# Autodesk Inventor assembly: Upper Stage
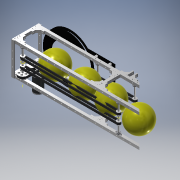
[picture p0: Inventor's stored thumbnail of the model, 180x180]
Saved by Autodesk Inventor 2019.4 (Build 234330000, 330)
## iProperties
Created: 2020-01-18
Part Number: Upper Stage
Document SubType Name: Assembly
Designer: Mark
Mass: 13649.7 g
Surface Area: 29206.4 cm^2
Volume: 17282.3 cm^3
Density: 0.789809 g/cm^3
Author: Mark
## Documents named in this file (21)
- C:\Users\admin\Desktop\FRC 2020 Engineering\GitHub\7738-2020\Upper Stage\Upper Stage.iam
- C:\Users\admin\Desktop\FRC 2020 Engineering\GitHub\7738-2020\Upper Stage\Main Extrusions.ipt
- C:\Users\admin\Desktop\FRC 2020 Engineering\GitHub\7738-2020\Upper Stage\Secondary Extrusions.ipt
- C:\Users\admin\Desktop\FRC 2020 Engineering\GitHub\7738-2020\Power Cell.ipt
- C:\Users\admin\Desktop\FRC 2020 Engineering\GitHub\7738-2020\Upper Stage\First stage shaft.ipt
- C:\Users\admin\Desktop\FRC 2020 Engineering\GitHub\7738-2020\Upper Stage\KFL08.ipt
- C:\Users\admin\Desktop\FRC 2020 Engineering\GitHub\7738-2020\Upper Stage\Turret Support.ipt
- C:\Users\admin\Desktop\FRC 2020 Engineering\GitHub\7738-2020\Upper Stage\HTD 5M 15 Teeth.ipt
- C:\Users\admin\Desktop\FRC 2020 Engineering\GitHub\7738-2020\Upper Stage\HTD 5M 775.ipt
- C:\Users\admin\Desktop\FRC 2020 Engineering\GitHub\7738-2020\Upper Stage\Turret Support 2.ipt
- C:\Users\admin\Desktop\FRC 2020 Engineering\GitHub\7738-2020\Upper Stage\Side Plates.ipt
- C:\Users\admin\Desktop\FRC 2020 Engineering\GitHub\7738-2020\Upper Stage\Vertical Support 1.ipt
- C:\Users\admin\Desktop\FRC 2020 Engineering\GitHub\7738-2020\Upper Stage\Back Brace.ipt
- C:\Users\admin\Desktop\FRC 2020 Engineering\GitHub\7738-2020\Upper Stage\Small Support.ipt
- C:\Users\admin\Desktop\FRC 2020 Engineering\GitHub\7738-2020\Upper Stage\Back Shaft.ipt
- C:\Users\admin\Desktop\FRC 2020 Engineering\GitHub\7738-2020\Upper Stage\Long Belt.ipt
- C:\Users\admin\Desktop\FRC 2020 Engineering\GitHub\7738-2020\Upper Stage\am-0255 2.5inch CIM Motor.ipt
- C:\Users\admin\Desktop\FRC 2020 Engineering\GitHub\7738-2020\Upper Stage\Motor Plate.ipt
- C:\Users\admin\Desktop\FRC 2020 Engineering\GitHub\7738-2020\Upper Stage\HTD 5M 40 Teeth.ipt
- C:\Users\admin\Desktop\FRC 2020 Engineering\GitHub\7738-2020\Upper Stage\Short First Stage Belt.ipt
- C:\Users\admin\Desktop\FRC 2020 Engineering\GitHub\7738-2020\Elevator Mechanism\Standard Bracing.ipt
## Components (62 placed, 20 different names)
1. Main Extrusions:1 — Mate:1, Flush:1, Flush:2, Flush:8, Mate:48, Mate:49, Mate:50, Mate:54, Mate:55, Mate:56, Mate:96, Flush:39, Mate:114, Mate:115, Flush:50, Mate:116, Mate:117, Flush:51, Mate:120, Mate:121, Flush:53
2. Main Extrusions:2 — Mate:1, Flush:1, Flush:2, Flush:5, Flush:7, Mate:3, Flush:20, Flush:21, Mate:39, Mate:40, Mate:41, Flush:31, Mate:45, Mate:46, Mate:47, Mate:51, Mate:52, Mate:53, Flush:41, Mate:106, Mate:107, Flush:46, Mate:108, Mate:109, Flush:47, Mate:118, Mate:119, Flush:52
3. Secondary Extrusions:1 — Flush:5, Flush:7, Flush:9, Mate:3, Mate:4, Mate:5, Mate:6, Mate:13, Mate:14, Mate:15, Flush:15, Mate:35, Mate:36, Mate:42, Flush:32, Mate:43, Mate:66, Mate:67, Mate:68, Mate:69, Mate:97, Mate:98, Mate:99, Flush:42, Mate:100, Mate:101, Flush:43, Mate:110, Mate:111, Flush:48, Mate:124, Flush:55, Mate:125
4. Secondary Extrusions:2 — Flush:8, Flush:9, Mate:7, Mate:8, Mate:9, Mate:10, Mate:11, Mate:12, Flush:14, Flush:15, Mate:62, Mate:63, Mate:64, Mate:65, Mate:102, Mate:103, Flush:44, Mate:104, Mate:105, Flush:45, Mate:122, Mate:123, Flush:54
5. Power Cell:1
6. Power Cell:2
7. Power Cell:3
8. Power Cell:4
9. First stage shaft:1 — Mate:16, Mate:17, Mate:22, Flush:12
10. KFL08:1 — Mate:4, Mate:5, Mate:6
11. KFL08:2 — Mate:7, Mate:8, Mate:9, Mate:16, Mate:17
12. KFL08:3 — Mate:13, Mate:14, Mate:15
13. KFL08:4 — Mate:10, Mate:11, Mate:12, Mate:18, Mate:19
14. First stage shaft:2 — Mate:18, Mate:19, Mate:23, Flush:13
15. Turret Support:1 — Mate:35, Mate:36, Mate:37, Mate:38
16. HTD 5M 15 Teeth:1 — Mate:22, Flush:12, Mate:24, Mate:61
17. HTD 5M 15 Teeth:2 — Mate:23, Flush:13, Mate:44
18. HTD 5M 775:1 — Mate:24, Mate:44, Mate:61
19. Turret Support 2:1 — Flush:14, Mate:37, Mate:38
20. Vertical Support 1:1 — Flush:20, Flush:21, Flush:22, Flush:23, Mate:32, Flush:28
21. Vertical Support 1:2 — Flush:22, Flush:23, Mate:32, Flush:26, Mate:34, Flush:27, Mate:39, Mate:77, Flush:33, Flush:40
22. Vertical Support 1:3 — Flush:28, Mate:112, Mate:113, Flush:49
23. Vertical Support 1:4 — Flush:26, Mate:34, Flush:27, Flush:38
24. Back Brace:1 — Mate:40, Mate:41, Flush:31
25. Back Brace:2 — Mate:42, Flush:32, Mate:43, Mate:78
26. KFL08:5 — Mate:45, Mate:46, Mate:47
27. KFL08:6 — Mate:48, Mate:49, Mate:50, Mate:57, Mate:58
28. KFL08:7 — Mate:51, Mate:52, Mate:53, Mate:70, Mate:84
29. KFL08:8 — Mate:54, Mate:55, Mate:56, Mate:71
30. First stage shaft:3 — Mate:57, Mate:58, Mate:59, Mate:93, Flush:37
31. HTD 5M 15 Teeth:3 — Mate:59, Mate:75, Mate:89, Flush:35, Mate:95, Flush:37
32. Small Support:1 — Mate:62, Mate:63
33. Small Support:2 — Mate:64, Mate:65
34. Small Support:3 — Mate:66, Mate:67
35. Small Support:4 — Mate:68, Mate:69
36. Back Shaft:1 — Mate:70, Mate:71, Mate:72, Mate:83, Mate:94
37. HTD 5M 15 Teeth:4 — Mate:72, Mate:74, Flush:35
38. Long Belt:1 — Mate:74, Mate:75, Mate:89
39. am-0255 2.5inch CIM Motor:1 — Mate:79, Mate:80, Mate:81, Mate:82
40. Motor Plate:1 — Mate:77, Flush:33, Mate:78, Mate:79, Mate:80, Mate:81
41. HTD 5M 40 Teeth:1 — Mate:83, Flush:34, Mate:84, Mate:86, Mate:88
42. HTD 5M 15 Teeth:5 — Mate:82, Flush:34, Mate:87
43. Short First Stage Belt:1 — Mate:85, Mate:86, Mate:87, Mate:88
44. HTD 5M 15 Teeth:6 — Mate:93, Mate:95
45. HTD 5M 15 Teeth:7 — Mate:94
46. Long Belt:2
47. Side Plates:1 — Mate:96, Flush:38, Flush:39
48. Side Plates:2 — Mate:97, Flush:40, Flush:41
49. Standard Bracing:1 — Mate:100, Mate:101, Flush:43
50. Standard Bracing:2 — Mate:106, Mate:107, Flush:46
51. Standard Bracing:3 — Mate:108, Mate:109, Flush:47
52. Standard Bracing:4 — Mate:110, Mate:111, Flush:48
53. Standard Bracing:5 — Mate:122, Mate:123, Flush:54
54. Standard Bracing:6 — Mate:120, Mate:121, Flush:53
55. Standard Bracing:7 — Mate:114, Mate:115, Flush:50
56. Standard Bracing:8 — Mate:98, Mate:99, Flush:42
57. Standard Bracing:9 — Mate:102, Mate:103, Flush:44
58. Standard Bracing:10 — Mate:104, Mate:105, Flush:45
59. Standard Bracing:11 — Mate:116, Mate:117, Flush:51
60. Standard Bracing:12 — Mate:118, Mate:119, Flush:52
61. Standard Bracing:13 — Mate:112, Mate:113, Flush:49
62. Standard Bracing:14 — Mate:124, Flush:55, Mate:125
## Relationships (155: Mate 111, Flush 44)
- Mate:1 (200 mm): Main Extrusions:1 ↔ Main Extrusions:2
- Flush:1: Main Extrusions:1 ↔ Main Extrusions:2
- Flush:2: Main Extrusions:1 ↔ Main Extrusions:2
- Flush:5: Main Extrusions:2 ↔ Secondary Extrusions:1
- Flush:7: Main Extrusions:2 ↔ Secondary Extrusions:1
- Flush:8: Main Extrusions:1 ↔ Secondary Extrusions:2
- Flush:9: Secondary Extrusions:1 ↔ Secondary Extrusions:2
- Mate:3 (150 mm): Main Extrusions:2 ↔ Secondary Extrusions:1
- Mate:4: Secondary Extrusions:1 ↔ KFL08:1
- Mate:5: Secondary Extrusions:1 ↔ KFL08:1
- Mate:6: Secondary Extrusions:1 ↔ KFL08:1
- Mate:7: Secondary Extrusions:2 ↔ KFL08:2
- Mate:8: Secondary Extrusions:2 ↔ KFL08:2
- Mate:9: Secondary Extrusions:2 ↔ KFL08:2
- Mate:10: Secondary Extrusions:2 ↔ KFL08:4
- Mate:11: Secondary Extrusions:2 ↔ KFL08:4
- Mate:12: Secondary Extrusions:2 ↔ KFL08:4
- Mate:13: Secondary Extrusions:1 ↔ KFL08:3
- Mate:14: Secondary Extrusions:1 ↔ KFL08:3
- Mate:15: Secondary Extrusions:1 ↔ KFL08:3
- Mate:16: First stage shaft:1 ↔ KFL08:2
- Mate:17 (0.2 mm): First stage shaft:1 ↔ KFL08:2
- Mate:18: KFL08:4 ↔ First stage shaft:2
- Mate:19 (0.2 mm): KFL08:4 ↔ First stage shaft:2
- Mate:22: First stage shaft:1 ↔ HTD 5M 15 Teeth:1
- Flush:12 (-9.5 mm): First stage shaft:1 ↔ HTD 5M 15 Teeth:1
- Mate:23: First stage shaft:2 ↔ HTD 5M 15 Teeth:2
- Flush:13 (-9.5 mm): First stage shaft:2 ↔ HTD 5M 15 Teeth:2
- Mate:24: HTD 5M 15 Teeth:1 ↔ HTD 5M 775:1
- Flush:14: Secondary Extrusions:2 ↔ Turret Support 2:1
- Flush:15: Secondary Extrusions:1 ↔ Secondary Extrusions:2
- Flush:20: Main Extrusions:2 ↔ Vertical Support 1:1
- Flush:21 (600 mm): Main Extrusions:2 ↔ Vertical Support 1:1
- Flush:22: Vertical Support 1:1 ↔ Vertical Support 1:2
- Flush:23: Vertical Support 1:1 ↔ Vertical Support 1:2
- Mate:32 (580 mm): Vertical Support 1:1 ↔ Vertical Support 1:2
- [Flush]: Vertical Support 1:3 ↔ Vertical Support 1:4
- [Flush]: Vertical Support 1:3 ↔ Vertical Support 1:4
- Flush:26: Vertical Support 1:2 ↔ Vertical Support 1:4
- Mate:34 (200 mm): Vertical Support 1:2 ↔ Vertical Support 1:4
- Flush:27: Vertical Support 1:2 ↔ Vertical Support 1:4
- Flush:28: Vertical Support 1:1 ↔ Vertical Support 1:3
- Mate:35: Secondary Extrusions:1 ↔ Turret Support:1
- Mate:36: Secondary Extrusions:1 ↔ Turret Support:1
- Mate:37: Turret Support:1 ↔ Turret Support 2:1
- Mate:38 (15.3 mm): Turret Support:1 ↔ Turret Support 2:1
- Mate:39: Main Extrusions:2 ↔ Vertical Support 1:2
- Mate:40: Main Extrusions:2 ↔ Back Brace:1
- Mate:41: Main Extrusions:2 ↔ Back Brace:1
- Flush:31: Main Extrusions:2 ↔ Back Brace:1
- Mate:42: Secondary Extrusions:1 ↔ Back Brace:2
- Flush:32: Secondary Extrusions:1 ↔ Back Brace:2
- Mate:43: Secondary Extrusions:1 ↔ Back Brace:2
- Mate:44: HTD 5M 15 Teeth:2 ↔ HTD 5M 775:1
- Mate:45: Main Extrusions:2 ↔ KFL08:5
- Mate:46: Main Extrusions:2 ↔ KFL08:5
- Mate:47: Main Extrusions:2 ↔ KFL08:5
- Mate:48: Main Extrusions:1 ↔ KFL08:6
- Mate:49: Main Extrusions:1 ↔ KFL08:6
- Mate:50: Main Extrusions:1 ↔ KFL08:6
- Mate:51: Main Extrusions:2 ↔ KFL08:7
- Mate:52: Main Extrusions:2 ↔ KFL08:7
- Mate:53: Main Extrusions:2 ↔ KFL08:7
- Mate:54: Main Extrusions:1 ↔ KFL08:8
- Mate:55: Main Extrusions:1 ↔ KFL08:8
- Mate:56: Main Extrusions:1 ↔ KFL08:8
- Mate:57: KFL08:6 ↔ First stage shaft:3
- Mate:58 (0.2 mm): KFL08:6 ↔ First stage shaft:3
- Mate:59: First stage shaft:3 ↔ HTD 5M 15 Teeth:3
- Mate:61 (0.5 mm): HTD 5M 15 Teeth:1 ↔ HTD 5M 775:1
- Mate:62: Secondary Extrusions:2 ↔ Small Support:1
- Mate:63: Secondary Extrusions:2 ↔ Small Support:1
- Mate:64: Secondary Extrusions:2 ↔ Small Support:2
- Mate:65: Secondary Extrusions:2 ↔ Small Support:2
- Mate:66: Secondary Extrusions:1 ↔ Small Support:3
- Mate:67: Secondary Extrusions:1 ↔ Small Support:3
- Mate:68: Secondary Extrusions:1 ↔ Small Support:4
- Mate:69: Secondary Extrusions:1 ↔ Small Support:4
- Mate:70: KFL08:7 ↔ Back Shaft:1
- Mate:71 (0.2 mm): KFL08:8 ↔ Back Shaft:1
- Mate:72: Back Shaft:1 ↔ HTD 5M 15 Teeth:4
- Mate:74: HTD 5M 15 Teeth:4 ↔ Long Belt:1
- Mate:75: HTD 5M 15 Teeth:3 ↔ Long Belt:1
- Mate:77: Vertical Support 1:2 ↔ Motor Plate:1
- Flush:33: Vertical Support 1:2 ↔ Motor Plate:1
- Mate:78: Back Brace:2 ↔ Motor Plate:1
- Mate:79: am-0255 2.5inch CIM Motor:1 ↔ Motor Plate:1
- Mate:80: am-0255 2.5inch CIM Motor:1 ↔ Motor Plate:1
- Mate:81: am-0255 2.5inch CIM Motor:1 ↔ Motor Plate:1
- Mate:82: am-0255 2.5inch CIM Motor:1 ↔ HTD 5M 15 Teeth:5
- Mate:83: Back Shaft:1 ↔ HTD 5M 40 Teeth:1
- Flush:34: HTD 5M 40 Teeth:1 ↔ HTD 5M 15 Teeth:5
- Mate:84 (1 mm): KFL08:7 ↔ HTD 5M 40 Teeth:1
- Mate:85: Short First Stage Belt:1
- Mate:86: HTD 5M 40 Teeth:1 ↔ Short First Stage Belt:1
- Mate:87: HTD 5M 15 Teeth:5 ↔ Short First Stage Belt:1
- Mate:88 (0.5 mm): HTD 5M 40 Teeth:1 ↔ Short First Stage Belt:1
- Mate:89 (0.5 mm): HTD 5M 15 Teeth:3 ↔ Long Belt:1
- Flush:35: HTD 5M 15 Teeth:3 ↔ HTD 5M 15 Teeth:4
- [Mate]: HTD 5M 15 Teeth:7 ↔ Long Belt:2
- [Mate]: HTD 5M 15 Teeth:6 ↔ Long Belt:2
- [Mate] (0.5 mm): HTD 5M 15 Teeth:6 ↔ Long Belt:2
- [Flush]: HTD 5M 15 Teeth:6 ↔ HTD 5M 15 Teeth:7
- Mate:93: First stage shaft:3 ↔ HTD 5M 15 Teeth:6
- Mate:94: Back Shaft:1 ↔ HTD 5M 15 Teeth:7
- Mate:95 (40 mm): HTD 5M 15 Teeth:3 ↔ HTD 5M 15 Teeth:6
- Flush:37 (-41 mm): First stage shaft:3 ↔ HTD 5M 15 Teeth:3
- Mate:96: Main Extrusions:1 ↔ Side Plates:1
- Flush:38: Vertical Support 1:4 ↔ Side Plates:1
- Flush:39: Main Extrusions:1 ↔ Side Plates:1
- Mate:97: Secondary Extrusions:1 ↔ Side Plates:2
- Flush:40: Vertical Support 1:2 ↔ Side Plates:2
- Flush:41: Main Extrusions:2 ↔ Side Plates:2
- Mate:98: Secondary Extrusions:1 ↔ Standard Bracing:8
- Mate:99: Secondary Extrusions:1 ↔ Standard Bracing:8
- Flush:42: Secondary Extrusions:1 ↔ Standard Bracing:8
- Mate:100: Secondary Extrusions:1 ↔ Standard Bracing:1
- Mate:101: Secondary Extrusions:1 ↔ Standard Bracing:1
- Flush:43: Secondary Extrusions:1 ↔ Standard Bracing:1
- Mate:102: Secondary Extrusions:2 ↔ Standard Bracing:9
- Mate:103: Secondary Extrusions:2 ↔ Standard Bracing:9
- Flush:44: Secondary Extrusions:2 ↔ Standard Bracing:9
- Mate:104: Secondary Extrusions:2 ↔ Standard Bracing:10
- Mate:105: Secondary Extrusions:2 ↔ Standard Bracing:10
- Flush:45: Secondary Extrusions:2 ↔ Standard Bracing:10
- Mate:106: Main Extrusions:2 ↔ Standard Bracing:2
- Mate:107: Main Extrusions:2 ↔ Standard Bracing:2
- Flush:46: Main Extrusions:2 ↔ Standard Bracing:2
- Mate:108: Main Extrusions:2 ↔ Standard Bracing:3
- Mate:109: Main Extrusions:2 ↔ Standard Bracing:3
- Flush:47: Main Extrusions:2 ↔ Standard Bracing:3
- Mate:110: Secondary Extrusions:1 ↔ Standard Bracing:4
- Mate:111: Secondary Extrusions:1 ↔ Standard Bracing:4
- Flush:48: Secondary Extrusions:1 ↔ Standard Bracing:4
- Mate:112: Vertical Support 1:3 ↔ Standard Bracing:13
- Mate:113: Vertical Support 1:3 ↔ Standard Bracing:13
- Flush:49: Vertical Support 1:3 ↔ Standard Bracing:13
- Mate:114: Main Extrusions:1 ↔ Standard Bracing:7
- Mate:115: Main Extrusions:1 ↔ Standard Bracing:7
- Flush:50: Main Extrusions:1 ↔ Standard Bracing:7
- Mate:116: Main Extrusions:1 ↔ Standard Bracing:11
- Mate:117: Main Extrusions:1 ↔ Standard Bracing:11
- Flush:51: Main Extrusions:1 ↔ Standard Bracing:11
- Mate:118: Main Extrusions:2 ↔ Standard Bracing:12
- Mate:119: Main Extrusions:2 ↔ Standard Bracing:12
- Flush:52: Main Extrusions:2 ↔ Standard Bracing:12
- Mate:120: Main Extrusions:1 ↔ Standard Bracing:6
- Mate:121: Main Extrusions:1 ↔ Standard Bracing:6
- Flush:53: Main Extrusions:1 ↔ Standard Bracing:6
- Mate:122: Secondary Extrusions:2 ↔ Standard Bracing:5
- Mate:123: Secondary Extrusions:2 ↔ Standard Bracing:5
- Flush:54: Secondary Extrusions:2 ↔ Standard Bracing:5
- Mate:124: Secondary Extrusions:1 ↔ Standard Bracing:14
- Flush:55: Secondary Extrusions:1 ↔ Standard Bracing:14
- Mate:125: Secondary Extrusions:1 ↔ Standard Bracing:14
## Named parameters: d56_d53 = 0 mm, d57_d54 = 0 mm, d143_d119 = 0 mm, d144_d120 = 0 mm, d145_d141 = 0.5 mm, d146_d142 = 0 mm
